# Autodesk Inventor assembly: GearExample
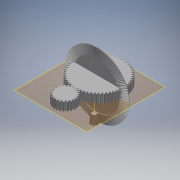
[picture p0: Inventor's stored thumbnail of the model, 180x180]
Saved by Autodesk Inventor 2019.2 (Build 232265000, 265)
## iProperties
Created: 2018-12-29
Part Number: GearExample
Document SubType Name: Assembly
Designer: steele
Author: steele
## Documents named in this file (3)
- C:\git\CAD-Development\robSteele\ShapeWays\GearExample.iam
- C:\git\CAD-Development\robSteele\ShapeWays\GearExample\Design Accelerator\Bevel Gears1.iam
- C:\git\CAD-Development\robSteele\ShapeWays\GearExample\Design Accelerator\Spur Gears1.iam
## Components (2 placed, 2 different names)
1. Bevel Gears:1 [sub-assembly] — Angle:1
2. Spur Gears:1 [sub-assembly] — Mate:1
## Relationships (2: Angle 1, Mate 1)
- Angle:1 (0 deg): Bevel Gears:1
- Mate:1: Spur Gears:1
